# Autodesk Inventor assembly: capflipper
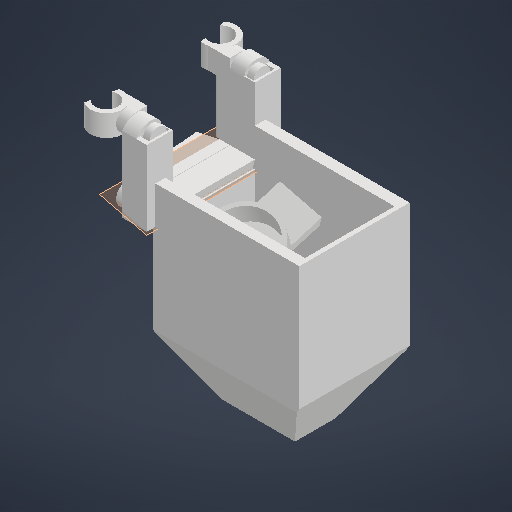
[picture p0: Inventor's stored thumbnail of the model, 512x512]
Saved by Autodesk Inventor 2026 (Build 300175050, 175E)
## iProperties
Created: 2026-05-08
Part Number: capflipper
Document SubType Name: Assembly
Designer: sniel
Author: sniel
## Documents named in this file (4)
- C:\Users\sniel\OneDrive\SDU\4_Semester\Applied automation\AppliedAutomationProject\feeder\capflipper.iam
- C:\Users\sniel\OneDrive\SDU\4_Semester\Applied automation\AppliedAutomationProject\feeder\capFlipperConnectionPoint.ipt
- C:\Users\sniel\OneDrive\SDU\4_Semester\Applied automation\AppliedAutomationProject\feeder\STEP\Wall v2\CapTurnerV1.ipt
- C:\Users\sniel\OneDrive\SDU\4_Semester\Applied automation\AppliedAutomationProject\feeder\Bottle.ipt
## Components (3 placed, 3 different names)
1. capFlipperConnectionPoint:1 — Mate:1, Mate:2, Mate:3
2. CapTurnerV1:1 — Mate:1, Mate:2, Mate:3, Mate:4
3. Bottle:1 — Mate:4
## Relationships (4: Mate 4)
- Mate:1: capFlipperConnectionPoint:1 ↔ CapTurnerV1:1
- Mate:2: capFlipperConnectionPoint:1 ↔ CapTurnerV1:1
- Mate:3 (0.25 mm): capFlipperConnectionPoint:1 ↔ CapTurnerV1:1
- Mate:4: CapTurnerV1:1 ↔ Bottle:1
